# Autodesk Inventor assembly: am-3563 4IN 8mm Round Compliant Wheel
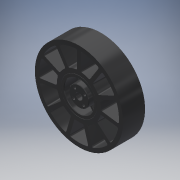
[picture p0: Inventor's stored thumbnail of the model, 180x180]
Saved by Autodesk Inventor 2019 (Build 230136000, 136)
## iProperties
Created: 2017-05-15
Part Number: am-3563 4IN 8mm Round Compliant Wheel
Description: STEP AP214
Document SubType Name: Assembly
Designer: josh
Sending System: SolidWorks 2017
Preprocessor: SwSTEP 2.0
Title: am-3563 4IN Compliant Wheel 8mm Round.STEP
Revision Number: ANY
## Documents named in this file (3)
- D:\Synthesis Robots\Epsilon\Epsilon Grabbers\am-3563 4IN 8mm Round Compliant Wheel.iam
- D:\Synthesis Robots\Epsilon\Epsilon Grabbers\4IN Compliant Wheel FINAL Overmold.ipt
- D:\Synthesis Robots\Epsilon\Epsilon Grabbers\2in Wheel Intergrated 8mm Hub.ipt
## Components (2 placed, 2 different names)
1. 4IN Compliant Wheel FINAL Overmold_1 — Mate:1, Flush:1
2. 2in Wheel Intergrated 8mm Hub_2 — Mate:1, Flush:1
## Relationships (2: Mate 1, Flush 1)
- Mate:1: 4IN Compliant Wheel FINAL Overmold_1 ↔ 2in Wheel Intergrated 8mm Hub_2
- Flush:1: 4IN Compliant Wheel FINAL Overmold_1 ↔ 2in Wheel Intergrated 8mm Hub_2
